# Autodesk Inventor assembly: TCRT5000L Module
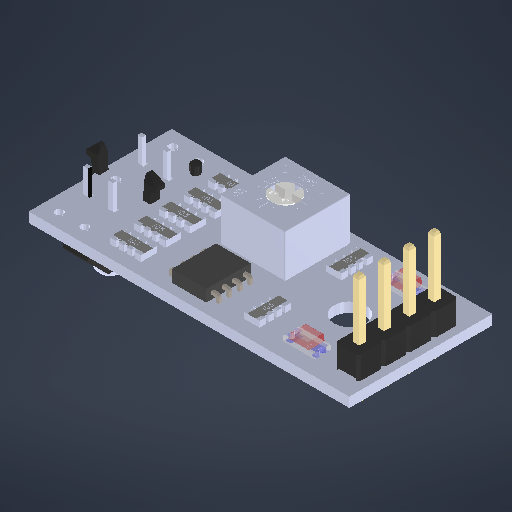
[picture p0: Inventor's stored thumbnail of the model, 512x512]
Saved by Autodesk Inventor 2026.1 (Build 301233020, 233B)
## iProperties
Created: 2017-09-16
Part Number: TCRT5000L Module
Description: SolidWorks IGES file using analytic representation for surfaces
Document SubType Name: Assembly
Designer: celio
Sending System: SolidWorks 2016
Preprocessor: SolidWorks 2016
Minimum Resolution: 0.0
Sending System Product ID: Assem2
Receiving System Product ID: Assem2
Sent Units: Millimeter
Translation Standard: IGES 5.3
Model Creation Time: 2017-09-16
Title: C:\Users\mohammad\Desktop\TCRT5000L Module.IGS
Author: mohammad
## Documents named in this file (11)
- C:\Users\celio\OneDrive\Documentos\Inventor\ZeGuia\Sensores\TCRT5000\TCRT5000.iam
- C:\Users\celio\OneDrive\Documentos\Inventor\ZeGuia\Sensores\TCRT5000\parts\Board.ipt
- C:\Users\celio\OneDrive\Documentos\Inventor\ZeGuia\Sensores\TCRT5000\parts\LEDs.ipt
- C:\Users\celio\OneDrive\Documentos\Inventor\ZeGuia\Sensores\TCRT5000\parts\Metal Contacts.ipt
- C:\Users\celio\OneDrive\Documentos\Inventor\ZeGuia\Sensores\TCRT5000\parts\TCRT50003.ipt
- C:\Users\celio\OneDrive\Documentos\Inventor\ZeGuia\Sensores\TCRT5000\parts\Pin Header.ipt
- C:\Users\celio\OneDrive\Documentos\Inventor\ZeGuia\Sensores\TCRT5000\parts\3362P-1-102LF-final.ipt
- C:\Users\celio\OneDrive\Documentos\Inventor\ZeGuia\Sensores\TCRT5000\parts\LM393 IC.ipt
- C:\Users\celio\OneDrive\Documentos\Inventor\ZeGuia\Sensores\TCRT5000\parts\103 SMD.ipt
- C:\Users\celio\OneDrive\Documentos\Inventor\ZeGuia\Sensores\TCRT5000\parts\Surface Mount Chip LED 3.2x1.6mm 2.ipt
- C:\Users\celio\OneDrive\Documentos\Inventor\ZeGuia\Pinos\Macho\1x4\1x4.iam
## Components (17 placed, 10 different names)
1. Board — Rígida:1
2. LEDs
3. Metal Contacts
4. TCRT50003
5. Pin Header
6. 3362P-1-102LF-final
7. LM393 IC
8. 103 SMD
9. 103 SMD:1
10. 103 SMD:2
11. 103 SMD:3
12. 103 SMD:4
13. 103 SMD:5
14. 103 SMD:6
15. Surface Mount Chip LED 3.2x1.6mm 2
16. Surface Mount Chip LED 3.2x1.6mm 2:1
17. 1x4:1 [sub-assembly] — Rígida:1
## Relationships (1: WeldJoint 1)
- Rígida:1 [WeldJoint] (-2.8 mm): Board ↔ 1x4:1
